# Autodesk Inventor assembly: CARCASA_ESTRUCTURA_Y_CHAPAS
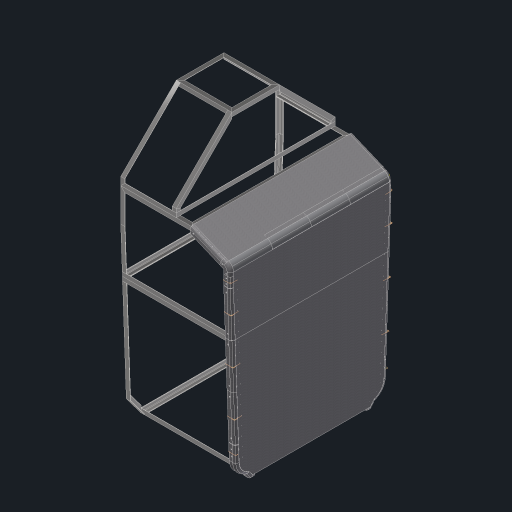
[picture p0: Inventor's stored thumbnail of the model, 512x512]
Saved by Autodesk Inventor 2024.3 (Build 283343000, 343)
## iProperties
Created: 2024-05-18
Part Number: CARCASA_ESTRUCTURA_Y_CHAPAS
Material: Generic
Document SubType Name: Assembly
Designer: Niler
Author: Niler
## Documents named in this file (21)
- C:\Users\Niler\OneDrive\Escritorio\RECICLADOR\RECICLADOR_MODELO_3D\VERSION_3_COMPLETA\CARCASA_ESTRUCTURA_Y_CHAPAS.iam
- C:\Users\Niler\OneDrive\Escritorio\RECICLADOR\RECICLADOR_MODELO_3D\VERSION_3_COMPLETA\ESTRUCTURA\ESTRUCTURA_COMPLETA.iam
- C:\Users\Niler\OneDrive\Escritorio\RECICLADOR\RECICLADOR_MODELO_3D\VERSION_3_COMPLETA\ESQUINAS\ESQUINA_REDONDEADA_R20_P1.ipt
- C:\Users\Niler\OneDrive\Escritorio\RECICLADOR\RECICLADOR_MODELO_3D\VERSION_3_COMPLETA\ESQUINAS\ESQUINA_REDONDEADA_R20_P2.ipt
- C:\Users\Niler\OneDrive\Escritorio\RECICLADOR\RECICLADOR_MODELO_3D\VERSION_3_COMPLETA\ESQUINAS\ESQUINA_REDONDEADA_R20_P3.ipt
- C:\Users\Niler\OneDrive\Escritorio\RECICLADOR\RECICLADOR_MODELO_3D\VERSION_3_COMPLETA\ESQUINAS\ESQUINA_REDONDEADA_R50.ipt
- C:\Users\Niler\OneDrive\Escritorio\RECICLADOR\RECICLADOR_MODELO_3D\VERSION_3_COMPLETA\ESQUINAS\ESQUINA_REDONDEADA_R50_P2.ipt
- C:\Users\Niler\OneDrive\Escritorio\RECICLADOR\RECICLADOR_MODELO_3D\VERSION_3_COMPLETA\ESQUINAS\ESQUINA_REDONDEADA_R20_P1_MIR.ipt
- C:\Users\Niler\OneDrive\Escritorio\RECICLADOR\RECICLADOR_MODELO_3D\VERSION_3_COMPLETA\ESQUINAS\ESQUINA_REDONDEADA_R20_P2_MIR.ipt
- C:\Users\Niler\OneDrive\Escritorio\RECICLADOR\RECICLADOR_MODELO_3D\VERSION_3_COMPLETA\ESQUINAS\ESQUINA_REDONDEADA_R20_P3_MIR.ipt
- C:\Users\Niler\OneDrive\Escritorio\RECICLADOR\RECICLADOR_MODELO_3D\VERSION_3_COMPLETA\ESQUINAS\ESQUINA_REDONDEADA_R20_P4.ipt
- C:\Users\Niler\OneDrive\Escritorio\RECICLADOR\RECICLADOR_MODELO_3D\VERSION_3_COMPLETA\ESQUINAS\ESQUINA_REDONDEADA_R20_P5.ipt
- C:\Users\Niler\OneDrive\Escritorio\RECICLADOR\RECICLADOR_MODELO_3D\VERSION_3_COMPLETA\ESQUINAS\ESQUINA_REDONDEADA_R20_P8.ipt
- C:\Users\Niler\OneDrive\Escritorio\RECICLADOR\RECICLADOR_MODELO_3D\VERSION_3_COMPLETA\ESQUINAS\ESQUINA_REDONDEADA_R20_P9.ipt
- C:\Users\Niler\OneDrive\Escritorio\RECICLADOR\RECICLADOR_MODELO_3D\VERSION_3_COMPLETA\ESQUINAS\ESQUINA_REDONDEADA_R20_P4_MIR.ipt
- C:\Users\Niler\OneDrive\Escritorio\RECICLADOR\RECICLADOR_MODELO_3D\VERSION_3_COMPLETA\ESQUINAS\ESQUINA_REDONDEADA_R20_P5_MIR.ipt
- C:\Users\Niler\OneDrive\Escritorio\RECICLADOR\RECICLADOR_MODELO_3D\VERSION_3_COMPLETA\ESQUINAS\ESQUINA_REDONDEADA_R20_P8_MIR.ipt
- C:\Users\Niler\OneDrive\Escritorio\RECICLADOR\RECICLADOR_MODELO_3D\VERSION_3_COMPLETA\ESQUINAS\ESQUINA_REDONDEADA_R20_P9_MIR.ipt
- C:\Users\Niler\OneDrive\Escritorio\RECICLADOR\RECICLADOR_MODELO_3D\VERSION_3_COMPLETA\NUEVAS_CHAPAS_ALUMINIO\CHAPA_1.ipt
- C:\Users\Niler\OneDrive\Escritorio\RECICLADOR\RECICLADOR_MODELO_3D\VERSION_3_COMPLETA\NUEVAS_CHAPAS_ALUMINIO\CHAPA_2.ipt
- C:\Users\Niler\OneDrive\Escritorio\RECICLADOR\RECICLADOR_MODELO_3D\VERSION_3_COMPLETA\NUEVAS_CHAPAS_ALUMINIO\CHAPA_3.ipt
## Components (38 placed, 20 different names)
1. ESTRUCTURA_COMPLETA:1 [sub-assembly] — Mate:2, Angle:1, Mate:3, Angle:2, Mate:9, Mate:10, Mate:11, Mate:16, Mate:17, Mate:22, Mate:23, Mate:24, Mate:25, Mate:31, Mate:38, Mate:39, Mate:41, Mate:46, Mate:47, Mate:48, Mate:54, Mate:55, Mate:56
2. ESQUINA_REDONDEADA_R20_P1:1 — Mate:2, Angle:1, Mate:4, Mate:30
3. ESQUINA_REDONDEADA_R20_P2:1 — Mate:3, Angle:2, Mate:4, Mate:29, Mate:72, Mate:73
4. ESQUINA_REDONDEADA_R20_P3:1 — Mate:9, Mate:10, Mate:11, Flush:2, Flush:3, Flush:4, Mate:29, Mate:30, Mate:32, Flush:6, Mate:42, Mate:76
5. ESQUINA_REDONDEADA_R50:1 — Flush:2, Mate:74
6. ESQUINA_REDONDEADA_R50_P2:1 — Flush:3, Flush:4, Mate:27, Mate:75
7. ESQUINA_REDONDEADA_R20_P1_MIR:1 — Flush:5, Mate:13
8. ESQUINA_REDONDEADA_R20_P2_MIR:1 — Flush:5, Mate:13
9. ESQUINA_REDONDEADA_R20_P3_MIR:1
10. ESQUINA_REDONDEADA_R50:2 — Mate:14, Mate:15, Mate:16
11. ESQUINA_REDONDEADA_R50_P2:2 — Mate:14, Mate:15, Mate:17, Mate:27, Mate:28
12. ESQUINA_REDONDEADA_R50:3 — Mate:23, Mate:26
13. ESQUINA_REDONDEADA_R50_P2:3 — Mate:22, Mate:28
14. ESQUINA_REDONDEADA_R50:4 — Mate:24, Mate:26
15. ESQUINA_REDONDEADA_R50_P2:4 — Mate:25
16. ESQUINA_REDONDEADA_R20_P4:1 — Mate:31, Mate:32, Flush:6, Mate:40
17. ESQUINA_REDONDEADA_R20_P5:1 — Mate:35, Mate:36, Mate:37, Mate:38
18. ESQUINA_REDONDEADA_R20_P5:2 — Mate:35, Mate:36, Mate:37, Mate:39, Mate:49
19. ESQUINA_REDONDEADA_R20_P4:2 — Mate:40, Mate:41, Mate:42, Mate:49
20. ESQUINA_REDONDEADA_R20_P5:3 — Mate:47, Mate:48, Flush:8, Mate:53
21. ESQUINA_REDONDEADA_R20_P5:4 — Mate:46, Flush:7
22. ESQUINA_REDONDEADA_R20_P5:5 — Flush:8, Mate:53, Flush:9
23. ESQUINA_REDONDEADA_R20_P5:6 — Flush:7, Flush:10, Mate:78
24. ESQUINA_REDONDEADA_R20_P8:1 — Mate:54, Flush:9, Mate:55, Mate:57
25. ESQUINA_REDONDEADA_R20_P9:1 — Mate:56, Flush:10, Mate:57
26. ESQUINA_REDONDEADA_R20_P4_MIR:1 — Mate:62
27. ESQUINA_REDONDEADA_R20_P5_MIR:1 — Mate:58, Mate:59, Mate:60
28. ESQUINA_REDONDEADA_R20_P5_MIR:2 — Mate:58, Mate:59, Mate:60, Mate:61, Mate:77
29. ESQUINA_REDONDEADA_R20_P4_MIR:2 — Mate:61, Mate:62
30. ESQUINA_REDONDEADA_R20_P5_MIR:3 — Mate:63, Mate:64, Mate:65, Mate:66, Flush:11
31. ESQUINA_REDONDEADA_R20_P5_MIR:4 — Mate:63, Mate:64, Mate:65, Flush:12, Mate:80
32. ESQUINA_REDONDEADA_R20_P5_MIR:5 — Mate:66, Flush:11, Mate:67, Mate:68, Mate:69, Flush:13
33. ESQUINA_REDONDEADA_R20_P5_MIR:6 — Flush:12, Mate:67, Mate:68, Mate:69, Flush:14
34. ESQUINA_REDONDEADA_R20_P8_MIR:1 — Flush:13, Mate:70
35. ESQUINA_REDONDEADA_R20_P9_MIR:1 — Mate:70, Flush:14
36. CHAPA_1:1 — Mate:72, Mate:73, Mate:74
37. CHAPA_2:1 — Mate:75, Mate:76, Mate:77, Mate:79
38. CHAPA_3:1 — Mate:78, Mate:79, Mate:80
## Relationships (86: Mate 71, Flush 13, Angle 2)
- Mate:2: ESTRUCTURA_COMPLETA:1 ↔ ESQUINA_REDONDEADA_R20_P1:1
- Angle:1 (0 deg): ESTRUCTURA_COMPLETA:1 ↔ ESQUINA_REDONDEADA_R20_P1:1
- Mate:3: ESTRUCTURA_COMPLETA:1 ↔ ESQUINA_REDONDEADA_R20_P2:1
- Angle:2 (0 deg): ESTRUCTURA_COMPLETA:1 ↔ ESQUINA_REDONDEADA_R20_P2:1
- Mate:4: ESQUINA_REDONDEADA_R20_P1:1 ↔ ESQUINA_REDONDEADA_R20_P2:1
- Mate:9: ESTRUCTURA_COMPLETA:1 ↔ ESQUINA_REDONDEADA_R20_P3:1
- Mate:10: ESTRUCTURA_COMPLETA:1 ↔ ESQUINA_REDONDEADA_R20_P3:1
- Mate:11: ESTRUCTURA_COMPLETA:1 ↔ ESQUINA_REDONDEADA_R20_P3:1
- Flush:2: ESQUINA_REDONDEADA_R20_P3:1 ↔ ESQUINA_REDONDEADA_R50:1
- Flush:3: ESQUINA_REDONDEADA_R20_P3:1 ↔ ESQUINA_REDONDEADA_R50_P2:1
- Flush:4: ESQUINA_REDONDEADA_R20_P3:1 ↔ ESQUINA_REDONDEADA_R50_P2:1
- Flush:5: ESQUINA_REDONDEADA_R20_P1_MIR:1 ↔ ESQUINA_REDONDEADA_R20_P2_MIR:1
- Mate:13: ESQUINA_REDONDEADA_R20_P1_MIR:1 ↔ ESQUINA_REDONDEADA_R20_P2_MIR:1
- Mate:14: ESQUINA_REDONDEADA_R50:2 ↔ ESQUINA_REDONDEADA_R50_P2:2
- Mate:15: ESQUINA_REDONDEADA_R50:2 ↔ ESQUINA_REDONDEADA_R50_P2:2
- Mate:16: ESTRUCTURA_COMPLETA:1 ↔ ESQUINA_REDONDEADA_R50:2
- Mate:17: ESTRUCTURA_COMPLETA:1 ↔ ESQUINA_REDONDEADA_R50_P2:2
- [Mate]: ESQUINA_REDONDEADA_R50:3 ↔ ESQUINA_REDONDEADA_R50_P2:3
- [Mate]: ESQUINA_REDONDEADA_R50:3 ↔ ESQUINA_REDONDEADA_R50_P2:3
- [Mate]: ESQUINA_REDONDEADA_R50:4 ↔ ESQUINA_REDONDEADA_R50_P2:4
- [Mate]: ESQUINA_REDONDEADA_R50:4 ↔ ESQUINA_REDONDEADA_R50_P2:4
- Mate:22: ESTRUCTURA_COMPLETA:1 ↔ ESQUINA_REDONDEADA_R50_P2:3
- Mate:23: ESTRUCTURA_COMPLETA:1 ↔ ESQUINA_REDONDEADA_R50:3
- Mate:24: ESTRUCTURA_COMPLETA:1 ↔ ESQUINA_REDONDEADA_R50:4
- Mate:25: ESTRUCTURA_COMPLETA:1 ↔ ESQUINA_REDONDEADA_R50_P2:4
- Mate:26: ESQUINA_REDONDEADA_R50:3 ↔ ESQUINA_REDONDEADA_R50:4
- Mate:27: ESQUINA_REDONDEADA_R50_P2:1 ↔ ESQUINA_REDONDEADA_R50_P2:2
- Mate:28: ESQUINA_REDONDEADA_R50_P2:2 ↔ ESQUINA_REDONDEADA_R50_P2:3
- Mate:29: ESQUINA_REDONDEADA_R20_P2:1 ↔ ESQUINA_REDONDEADA_R20_P3:1
- Mate:30: ESQUINA_REDONDEADA_R20_P1:1 ↔ ESQUINA_REDONDEADA_R20_P3:1
- Mate:31: ESTRUCTURA_COMPLETA:1 ↔ ESQUINA_REDONDEADA_R20_P4:1
- Mate:32: ESQUINA_REDONDEADA_R20_P3:1 ↔ ESQUINA_REDONDEADA_R20_P4:1
- Flush:6: ESQUINA_REDONDEADA_R20_P3:1 ↔ ESQUINA_REDONDEADA_R20_P4:1
- Mate:35: ESQUINA_REDONDEADA_R20_P5:1 ↔ ESQUINA_REDONDEADA_R20_P5:2
- Mate:36: ESQUINA_REDONDEADA_R20_P5:1 ↔ ESQUINA_REDONDEADA_R20_P5:2
- Mate:37: ESQUINA_REDONDEADA_R20_P5:1 ↔ ESQUINA_REDONDEADA_R20_P5:2
- Mate:38: ESTRUCTURA_COMPLETA:1 ↔ ESQUINA_REDONDEADA_R20_P5:1
- Mate:39: ESTRUCTURA_COMPLETA:1 ↔ ESQUINA_REDONDEADA_R20_P5:2
- Mate:40: ESQUINA_REDONDEADA_R20_P4:1 ↔ ESQUINA_REDONDEADA_R20_P4:2
- Mate:41: ESTRUCTURA_COMPLETA:1 ↔ ESQUINA_REDONDEADA_R20_P4:2
- Mate:42: ESQUINA_REDONDEADA_R20_P3:1 ↔ ESQUINA_REDONDEADA_R20_P4:2
- [Mate]: ESQUINA_REDONDEADA_R20_P5:3 ↔ ESQUINA_REDONDEADA_R20_P5:4
- [Mate]: ESQUINA_REDONDEADA_R20_P5:3 ↔ ESQUINA_REDONDEADA_R20_P5:4
- [Mate]: ESQUINA_REDONDEADA_R20_P5:3 ↔ ESQUINA_REDONDEADA_R20_P5:4
- Mate:46: ESTRUCTURA_COMPLETA:1 ↔ ESQUINA_REDONDEADA_R20_P5:4
- Mate:47: ESTRUCTURA_COMPLETA:1 ↔ ESQUINA_REDONDEADA_R20_P5:3
- Mate:48: ESTRUCTURA_COMPLETA:1 ↔ ESQUINA_REDONDEADA_R20_P5:3
- Mate:49: ESQUINA_REDONDEADA_R20_P5:2 ↔ ESQUINA_REDONDEADA_R20_P4:2
- [Mate]: ESQUINA_REDONDEADA_R20_P5:5 ↔ ESQUINA_REDONDEADA_R20_P5:6
- [Mate]: ESQUINA_REDONDEADA_R20_P5:5 ↔ ESQUINA_REDONDEADA_R20_P5:6
- [Mate]: ESQUINA_REDONDEADA_R20_P5:5 ↔ ESQUINA_REDONDEADA_R20_P5:6
- Flush:7: ESQUINA_REDONDEADA_R20_P5:4 ↔ ESQUINA_REDONDEADA_R20_P5:6
- Flush:8: ESQUINA_REDONDEADA_R20_P5:3 ↔ ESQUINA_REDONDEADA_R20_P5:5
- Mate:53: ESQUINA_REDONDEADA_R20_P5:3 ↔ ESQUINA_REDONDEADA_R20_P5:5
- Mate:54: ESTRUCTURA_COMPLETA:1 ↔ ESQUINA_REDONDEADA_R20_P8:1
- Flush:9: ESQUINA_REDONDEADA_R20_P5:5 ↔ ESQUINA_REDONDEADA_R20_P8:1
- Mate:55: ESTRUCTURA_COMPLETA:1 ↔ ESQUINA_REDONDEADA_R20_P8:1
- Mate:56: ESTRUCTURA_COMPLETA:1 ↔ ESQUINA_REDONDEADA_R20_P9:1
- Flush:10: ESQUINA_REDONDEADA_R20_P5:6 ↔ ESQUINA_REDONDEADA_R20_P9:1
- Mate:57: ESQUINA_REDONDEADA_R20_P8:1 ↔ ESQUINA_REDONDEADA_R20_P9:1
- Mate:58: ESQUINA_REDONDEADA_R20_P5_MIR:1 ↔ ESQUINA_REDONDEADA_R20_P5_MIR:2
- Mate:59: ESQUINA_REDONDEADA_R20_P5_MIR:1 ↔ ESQUINA_REDONDEADA_R20_P5_MIR:2
- Mate:60: ESQUINA_REDONDEADA_R20_P5_MIR:1 ↔ ESQUINA_REDONDEADA_R20_P5_MIR:2
- Mate:61: ESQUINA_REDONDEADA_R20_P5_MIR:2 ↔ ESQUINA_REDONDEADA_R20_P4_MIR:2
- Mate:62: ESQUINA_REDONDEADA_R20_P4_MIR:1 ↔ ESQUINA_REDONDEADA_R20_P4_MIR:2
- Mate:63: ESQUINA_REDONDEADA_R20_P5_MIR:3 ↔ ESQUINA_REDONDEADA_R20_P5_MIR:4
- Mate:64: ESQUINA_REDONDEADA_R20_P5_MIR:3 ↔ ESQUINA_REDONDEADA_R20_P5_MIR:4
- Mate:65: ESQUINA_REDONDEADA_R20_P5_MIR:3 ↔ ESQUINA_REDONDEADA_R20_P5_MIR:4
- Mate:66: ESQUINA_REDONDEADA_R20_P5_MIR:3 ↔ ESQUINA_REDONDEADA_R20_P5_MIR:5
- Flush:11: ESQUINA_REDONDEADA_R20_P5_MIR:3 ↔ ESQUINA_REDONDEADA_R20_P5_MIR:5
- Flush:12: ESQUINA_REDONDEADA_R20_P5_MIR:4 ↔ ESQUINA_REDONDEADA_R20_P5_MIR:6
- Mate:67: ESQUINA_REDONDEADA_R20_P5_MIR:5 ↔ ESQUINA_REDONDEADA_R20_P5_MIR:6
- Mate:68: ESQUINA_REDONDEADA_R20_P5_MIR:5 ↔ ESQUINA_REDONDEADA_R20_P5_MIR:6
- Mate:69: ESQUINA_REDONDEADA_R20_P5_MIR:5 ↔ ESQUINA_REDONDEADA_R20_P5_MIR:6
- Flush:13: ESQUINA_REDONDEADA_R20_P5_MIR:5 ↔ ESQUINA_REDONDEADA_R20_P8_MIR:1
- Mate:70: ESQUINA_REDONDEADA_R20_P8_MIR:1 ↔ ESQUINA_REDONDEADA_R20_P9_MIR:1
- Flush:14: ESQUINA_REDONDEADA_R20_P5_MIR:6 ↔ ESQUINA_REDONDEADA_R20_P9_MIR:1
- Mate:72: ESQUINA_REDONDEADA_R20_P2:1 ↔ CHAPA_1:1
- Mate:73: ESQUINA_REDONDEADA_R20_P2:1 ↔ CHAPA_1:1
- Mate:74: ESQUINA_REDONDEADA_R50:1 ↔ CHAPA_1:1
- Mate:75: ESQUINA_REDONDEADA_R50_P2:1 ↔ CHAPA_2:1
- Mate:76: ESQUINA_REDONDEADA_R20_P3:1 ↔ CHAPA_2:1
- Mate:77: ESQUINA_REDONDEADA_R20_P5_MIR:2 ↔ CHAPA_2:1
- Mate:78: ESQUINA_REDONDEADA_R20_P5:6 ↔ CHAPA_3:1
- Mate:79: CHAPA_2:1 ↔ CHAPA_3:1
- Mate:80: ESQUINA_REDONDEADA_R20_P5_MIR:4 ↔ CHAPA_3:1
## Named parameters: d31_d27 = 0 mm, d32_d28 = 0 mm, d33_d27 = 0 mm, d34_d28 = 0 mm, d58_d50 = 0 mm, d59_d51 = 0 mm, d60_d52 = 0 mm, d65_d58_d50 = 0 mm, d66_d59_d51 = 0 mm, d67_d60_d52 = 0 mm
